# Autodesk Inventor assembly: Corner of Frame
Saved by Autodesk Inventor 2015 (Build 190159000, 159)
## iProperties
Created: 2015-01-11
Part Number: Corner of Frame
Document SubType Name: Assembly
Designer: jhirshland1
Author: jhirshland1
## Documents named in this file (3)
- C:\Users\jhirshland1\Inventor\HWRobot2015\Corner of Frame.iam
- C:\Users\jhirshland1\Inventor\HWRobot2015\FRCKOP2015\Drive Base\am-2951 AM14U2 Outside Sheet.ipt
- C:\Users\jhirshland1\Inventor\HWRobot2015\Imported Components\REV_simple_lift_pneumatics\REV-21-1002a.ipt
## Components (3 placed, 2 different names)
1. am-2951 AM14U2 Outside Sheet:1
2. am-2951 AM14U2 Outside Sheet:2
3. REV-21-1002a:1
## Relationships (3: Insert 3)
- [Insert]: am-2951 AM14U2 Outside Sheet:1 ↔ REV-21-1002a:1
- [Insert]: am-2951 AM14U2 Outside Sheet:1 ↔ REV-21-1002a:1
- [Insert]: am-2951 AM14U2 Outside Sheet:2 ↔ REV-21-1002a:1
